# Autodesk Inventor assembly: Lower Assembly
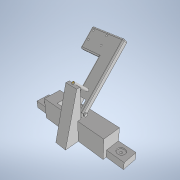
[picture p0: Inventor's stored thumbnail of the model, 180x180]
Saved by Autodesk Inventor 2020 (Build 240168000, 168)
## iProperties
Created: 2019-11-14
Part Number: Lower Assembly
Document SubType Name: Assembly
Designer: bzs3334
Author: bzs3334
## Documents named in this file (5)
- P:\GarbageGrader\Brackets\Lower Assembly.iam
- P:\GarbageGrader\Brackets\Bottom Bracket + camera bottom thingy.ipt
- P:\GarbageGrader\Brackets\fakeM4Bolt.ipt
- P:\GarbageGrader\Brackets\lever.ipt
- P:\GarbageGrader\Brackets\fakeM4BoltLonger.ipt
## Components (4 placed, 4 different names)
1. Bottom Bracket + camera bottom thingy:1 — Mate:1, Mate:2, Mate:7, Mate:8, Flush:1, Mate:10
2. fakeM4Bolt:1 — Mate:3, Mate:4
3. lever:1 — Mate:1, Mate:2, Mate:3, Mate:4, Mate:9
4. fakeM4BoltLonger:1 — Mate:9, Mate:10
## Relationships (9: Mate 8, Flush 1)
- Mate:1: Bottom Bracket + camera bottom thingy:1 ↔ lever:1
- Mate:2: Bottom Bracket + camera bottom thingy:1 ↔ lever:1
- Mate:3: fakeM4Bolt:1 ↔ lever:1
- Mate:4: fakeM4Bolt:1 ↔ lever:1
- Mate:7: Bottom Bracket + camera bottom thingy:1
- Mate:8: Bottom Bracket + camera bottom thingy:1
- Flush:1: Bottom Bracket + camera bottom thingy:1
- Mate:9: lever:1 ↔ fakeM4BoltLonger:1
- Mate:10: Bottom Bracket + camera bottom thingy:1 ↔ fakeM4BoltLonger:1
